# Autodesk Inventor assembly: Lidar Sensor Case Assembly Final
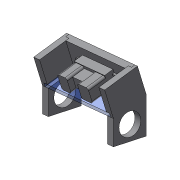
[picture p0: Inventor's stored thumbnail of the model, 180x180]
Saved by Autodesk Inventor 2018.3 (Build 223284000, 284)
## iProperties
Created: 2019-03-18
Part Number: Lidar Sensor Case Assembly Final
Document SubType Name: Assembly
Designer: aye06091
Mass: 28.7668 g
Surface Area: 168.728 cm^2
Volume: 28.7668 cm^3
Density: 1 g/cm^3
Author: aye06091
## Documents named in this file (6)
- Y:\DeSimony-R\Senior R&D\4 R&D Shared Folder\VisiStick\VisiStick (Inventor)\Physical Parts\Lidar Sensor Case Assembly Final.iam
- Y:\DeSimony-R\Senior R&D\4 R&D Shared Folder\VisiStick\VisiStick (Inventor)\Case Final\Lidar Sensor CAse Piece 1.ipt
- Y:\DeSimony-R\Senior R&D\4 R&D Shared Folder\VisiStick\VisiStick (Inventor)\Case Final\Lidar Sensor Case Piece 2.ipt
- Y:\DeSimony-R\Senior R&D\4 R&D Shared Folder\VisiStick\VisiStick (Inventor)\Case Final\Lidar Sensor Case Piece 3.ipt
- Y:\DeSimony-R\Senior R&D\4 R&D Shared Folder\VisiStick\VisiStick (Inventor)\Electronics\Sharp 2Y0A02.ipt
- Y:\DeSimony-R\Senior R&D\4 R&D Shared Folder\VisiStick\VisiStick (Inventor)\Physical Parts\Lidar Sensor Case 4 v2.ipt
## Components (5 placed, 5 different names)
1. Lidar Sensor CAse Piece 1:1 — Mate:1, Flush:1, Flush:2, Flush:3, Flush:4, Mate:3, Mate:4, Flush:5
2. Lidar Sensor Case Piece 2:1 — Flush:3, Flush:4, Mate:2
3. Lidar Sensor Case Piece 3:1 — Insert:1, Insert:2, Mate:1, Flush:1, Flush:2, Mate:2
4. Sharp 2Y0A02:1 — Insert:1, Insert:2
5. Lidar Sensor Case 4 v2:1 — Mate:3, Mate:4, Flush:5
## Relationships (11: Flush 5, Mate 4, Insert 2)
- Insert:1: Lidar Sensor Case Piece 3:1 ↔ Sharp 2Y0A02:1
- Insert:2: Lidar Sensor Case Piece 3:1 ↔ Sharp 2Y0A02:1
- Mate:1: Lidar Sensor CAse Piece 1:1 ↔ Lidar Sensor Case Piece 3:1
- Flush:1: Lidar Sensor CAse Piece 1:1 ↔ Lidar Sensor Case Piece 3:1
- Flush:2: Lidar Sensor CAse Piece 1:1 ↔ Lidar Sensor Case Piece 3:1
- Flush:3: Lidar Sensor CAse Piece 1:1 ↔ Lidar Sensor Case Piece 2:1
- Flush:4: Lidar Sensor CAse Piece 1:1 ↔ Lidar Sensor Case Piece 2:1
- Mate:2: Lidar Sensor Case Piece 2:1 ↔ Lidar Sensor Case Piece 3:1
- Mate:3: Lidar Sensor CAse Piece 1:1 ↔ Lidar Sensor Case 4 v2:1
- Mate:4: Lidar Sensor CAse Piece 1:1 ↔ Lidar Sensor Case 4 v2:1
- Flush:5: Lidar Sensor CAse Piece 1:1 ↔ Lidar Sensor Case 4 v2:1
